# Autodesk Inventor assembly: conjunto_engranes
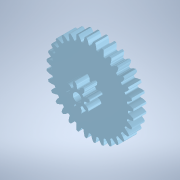
[picture p0: Inventor's stored thumbnail of the model, 180x180]
Saved by Autodesk Inventor 2022 (Build 260153000, 153)
## iProperties
Created: 2022-02-27
Part Number: conjunto_engranes
Document SubType Name: Assembly
Designer: Home
Author: Home
## Documents named in this file (3)
- C:\Users\Home\Dropbox\2022\DISEÑO E INNOVACIÓN  1\miniproyecto\conjunto_engranes.iam
- C:\Users\Home\Dropbox\2022\DISEÑO E INNOVACIÓN  1\miniproyecto\engranes_8dientes.ipt
- C:\Users\Home\Dropbox\2022\DISEÑO E INNOVACIÓN  1\miniproyecto\engrane_32dientes.ipt
## Components (2 placed, 2 different names)
1. engranes_8dientes:1 — Mate:1, Mate:2, Rotation:1
2. engrane_32dientes:1 — Mate:1, Mate:2, Rotation:1
## Relationships (3: Mate 2, RelateRotation 1)
- Mate:1: engranes_8dientes:1 ↔ engrane_32dientes:1
- Mate:2: engranes_8dientes:1 ↔ engrane_32dientes:1
- Rotation:1 [RelateRotation] (1 ul): engranes_8dientes:1 ↔ engrane_32dientes:1
